# Autodesk Inventor assembly: ramp
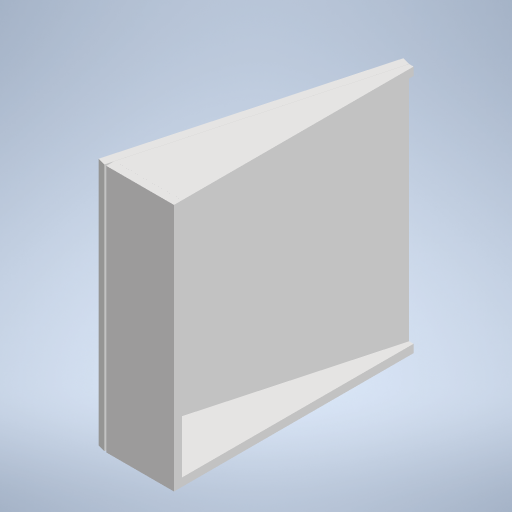
[picture p0: Inventor's stored thumbnail of the model, 512x512]
Saved by Autodesk Inventor 2024.2 (Build 282272000, 272)
## iProperties
Created: 2024-01-13
Part Number: ramp
Document SubType Name: Assembly
Designer: HukoOo
Author: HukoOo
## Documents named in this file (4)
- E:\OneDrive - 성균관대학교\Projects\2024 ICRA QRC 대회\모델\ramp.iam
- E:\OneDrive - 성균관대학교\Projects\2024 ICRA QRC 대회\모델\board_18x513x150.ipt
- E:\OneDrive - 성균관대학교\Projects\2024 ICRA QRC 대회\모델\board_18x550x150.ipt
- E:\OneDrive - 성균관대학교\Projects\2024 ICRA QRC 대회\모델\board_18x550x550.ipt
## Components (4 placed, 3 different names)
1. board_18x513x150:1 — 플러쉬:1, 플러쉬:4
2. board_18x550x150:1 — 플러쉬:1, 메이트:1, 플러쉬:2, 플러쉬:3
3. board_18x513x150:2 — 메이트:1, 플러쉬:2, 플러쉬:3
4. board_18x550x550:1 — 플러쉬:4
## Relationships (5: Flush 4, Mate 1)
- 플러쉬:1 [Flush]: board_18x513x150:1 ↔ board_18x550x150:1
- 메이트:1 [Mate]: board_18x550x150:1 ↔ board_18x513x150:2
- 플러쉬:2 [Flush]: board_18x550x150:1 ↔ board_18x513x150:2
- 플러쉬:3 [Flush]: board_18x550x150:1 ↔ board_18x513x150:2
- 플러쉬:4 [Flush]: board_18x513x150:1 ↔ board_18x550x550:1
